# Autodesk Inventor assembly: Electronics Box
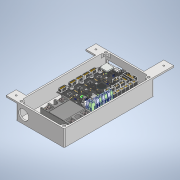
[picture p0: Inventor's stored thumbnail of the model, 180x180]
Saved by Autodesk Inventor 2022 (Build 260153000, 153)
## iProperties
Created: 2022-02-24
Part Number: Electronics Box
Document SubType Name: Assembly
Designer: Nick
Author: Nick
## Documents named in this file (4)
- Y:\Projects\Bibble0\Electronics Box.iam
- Y:\Projects\Bibble0\Electronics\SSR-40.ipt
- Y:\Projects\Bibble0\3D printed\Electronics Box.ipt
- Y:\Projects\Bibble0\SKR Mini E3 v2.0.ipt
## Components (3 placed, 3 different names)
1. Electronics Box:1 — Mate:2, Mate:3, Mate:4, Mate:5, Mate:7
2. SKR Mini E3 v2.0:1 — Mate:2, Mate:3, Mate:4, Mate:6
3. SSR-40:1 — Mate:5, Mate:6, Mate:7
## Relationships (6: Mate 6)
- Mate:2 (2 mm): Electronics Box:1 ↔ SKR Mini E3 v2.0:1
- Mate:3 (10 mm): Electronics Box:1 ↔ SKR Mini E3 v2.0:1
- Mate:4 (2 mm): Electronics Box:1 ↔ SKR Mini E3 v2.0:1
- Mate:5: Electronics Box:1 ↔ SSR-40:1
- Mate:6 (10 mm): SKR Mini E3 v2.0:1 ↔ SSR-40:1
- Mate:7 (5 mm): Electronics Box:1 ↔ SSR-40:1
